# Autodesk Inventor assembly: !Electronic Tray Assembly
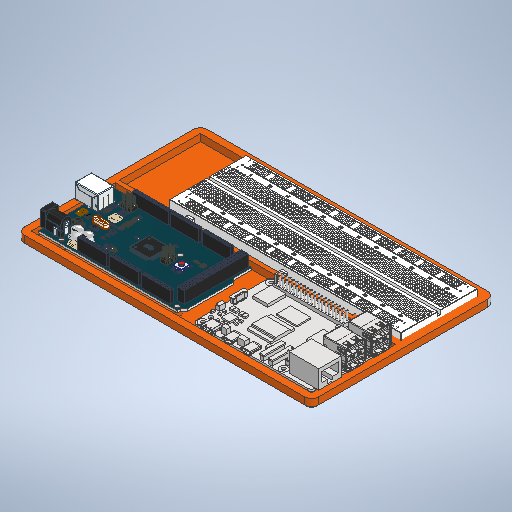
[picture p0: Inventor's stored thumbnail of the model, 512x512]
Saved by Autodesk Inventor 2025.2 (Build 292293000, 293)
## iProperties
Created: 2025-02-05
Part Number: !Electronic Tray Assembly
Document SubType Name: Assembly
Designer: caomi
Author: caomi
## Documents named in this file (5)
- C:\Minh Nguyen\H2A\cad\Misc Electronics\!Electronic Tray Assembly.iam
- C:\Minh Nguyen\H2A\cad\Misc Electronics\Electronic Base.ipt
- C:\Minh Nguyen\H2A\cad\Misc Electronics\RaspberryPi5.iam
- C:\Minh Nguyen\H2A\cad\Misc Electronics\Breadboard.ipt
- C:\Minh Nguyen\H2A\cad\Misc Electronics\arduino_MEGA2560\arduino_MEGA2560\arduino_MEGA2560.ipt
## Components (4 placed, 4 different names)
1. Electronic Base:1 — Rigid:1, Rigid:4, Rigid:5
2. RaspberryPi5:1 [sub-assembly] — Rigid:1
3. Breadboard:1 — Rigid:5
4. arduino_MEGA2560:1 — Rigid:4
## Relationships (3: WeldJoint 3)
- Rigid:1 [WeldJoint]: Electronic Base:1 ↔ RaspberryPi5:1
- Rigid:4 [WeldJoint]: Electronic Base:1 ↔ arduino_MEGA2560:1
- Rigid:5 [WeldJoint]: Electronic Base:1 ↔ Breadboard:1
